# Autodesk Inventor assembly: ControlHousing
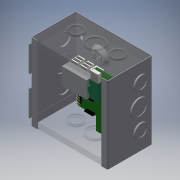
[picture p0: Inventor's stored thumbnail of the model, 180x180]
Saved by Autodesk Inventor 2016 (Build 200138000, 138)
## iProperties
Company: Unknown
Created: 2016-08-11
Part Number: ControlHousing
Description: Unknown
Document SubType Name: Assembly
Designer: jfixelle
Sending System: Unknown
Preprocessor: PSStep 14.0
Title: S:/STOCK/7-COMMERCIAL/CHKO/chko663.stp
Author: Unknown
Revision Number: NONE
## Documents named in this file (9)
- E:\jfixelle\Documents\APC\GitRepo\Control\IAM\ControlHousing.iam
- E:\jfixelle\Downloads\loc13368.ipt
- E:\jfixelle\Downloads\COM55083-4.ipt
- E:\jfixelle\Downloads\COM55563-4.ipt
- E:\jfixelle\Downloads\COM55989.ipt
- E:\jfixelle\Downloads\HNG11000.iam
- E:\jfixelle\Documents\APC\GitRepo\Control\IAM\PiB+.ipt
- E:\jfixelle\Documents\APC\GitRepo\Control\IAM\ControlBoard.iam
- E:\jfixelle\Documents\APC\GitRepo\Control\IAM\DB9Plug.ipt
## Components (10 placed, 10 different names)
1. NAUO4
2. NAUO5
3. NAUO6
4. NAUO7 — Mate:1, Mate:2
5. NAUO8
6. NAUO9 [sub-assembly]
7. NAUO10 [sub-assembly]
8. PiB+:1 — Mate:1
9. ControlBoard:1 [sub-assembly] — Mate:2, Flush:1, Mate:3, Flush:2
10. DB9Plug:1 — Flush:1, Mate:3, Flush:2
## Relationships (5: Mate 3, Flush 2)
- Mate:1 (11 mm): NAUO7 ↔ PiB+:1
- Mate:2 (38.1 mm): NAUO7 ↔ ControlBoard:1
- Flush:1 (-2.54 mm): ControlBoard:1 ↔ DB9Plug:1
- Mate:3: ControlBoard:1 ↔ DB9Plug:1
- Flush:2: ControlBoard:1 ↔ DB9Plug:1
